# Autodesk Inventor assembly: Montagem_Arduino
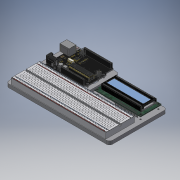
[picture p0: Inventor's stored thumbnail of the model, 180x180]
Saved by Autodesk Inventor 2017 (Build 210142000, 142)
## iProperties
Created: 2019-04-18
Part Number: Montagem_Arduino
Description: MONTAGEM TRABALHO
Document SubType Name: Assembly
Designer: Marcus
CONJUNTO: TEXTO CONJUNTO
EQUIPAMENTO: TEXTO EQUIPAMENTO
SUBCONJUNTO: TEXTO SUBCONJUNTO
Author: Marcus
## Documents named in this file (5)
- C:\Users\Marcus\Google Drive\Metal Class Projetos\Base Arduino\Montagem_Arduino.iam
- C:\Users\Marcus\Google Drive\Metal Class Projetos\Base Arduino\ArduinoUNO .ipt
- C:\Users\Marcus\Google Drive\Metal Class Projetos\Base Arduino\Plataforma.ipt
- C:\Users\Marcus\Google Drive\Metal Class Projetos\Base Arduino\LCD.ipt
- C:\Users\Marcus\Google Drive\Metal Class Projetos\Base Arduino\Protoboard.ipt
## Components (4 placed, 4 different names)
1. Plataforma:1 — Flush:7, Flush:8, Flush:9, Mate:1, Flush:10, Flush:11, Mate:2, Mate:3, Mate:4, Flush:13
2. ArduinoUNO :2 — Mate:1, Flush:10, Flush:11, Flush:12
3. LCD:1 — Mate:2, Flush:12, Mate:3
4. Protoboard:1 — Mate:4, Flush:13, Flush:14
## Relationships (12: Flush 8, Mate 4)
- Flush:7: Plataforma:1
- Flush:8: Plataforma:1
- Flush:9: Plataforma:1
- Mate:1 (3 mm): Plataforma:1 ↔ ArduinoUNO :2
- Flush:10 (2 mm): Plataforma:1 ↔ ArduinoUNO :2
- Flush:11 (5 mm): Plataforma:1 ↔ ArduinoUNO :2
- Mate:2: Plataforma:1 ↔ LCD:1
- Flush:12 (3 mm): ArduinoUNO :2 ↔ LCD:1
- Mate:3: Plataforma:1 ↔ LCD:1
- Mate:4: Plataforma:1 ↔ Protoboard:1
- Flush:13 (1 mm): Plataforma:1 ↔ Protoboard:1
- Flush:14: Protoboard:1
